# Autodesk Inventor assembly: roller
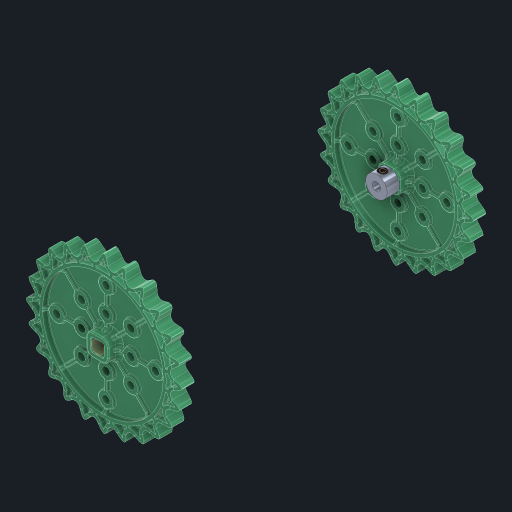
[picture p0: Inventor's stored thumbnail of the model, 512x512]
Saved by Autodesk Inventor 2024 (Build 280153000, 153)
## iProperties
Created: 2023-08-21
Part Number: roller
Document SubType Name: Assembly
Designer: Averey
Author: Averey
## Documents named in this file (4)
- C:\Users\Averey\Documents\vex\cad\scrap_v0.1\intake\roller.iam
- C:\Users\Averey\Documents\vex\cad\VEX-CAD-Inventor-1.41\Motion\Sprockets\9P Sprocket\9P 24T Sprocket, No Insert.iam
- C:\Users\Averey\Documents\vex\cad\VEX-CAD-Inventor-1.41\Motion\Sprockets\9P Sprocket.iam
- C:\Users\Averey\Documents\vex\cad\VEX-CAD-Inventor-1.41\Motion\Shaft LS\Shaft Collar ipts\Shaft Collar Set Screw.ipt
## Components (4 placed, 2 different names)
1. 9P 24T Sprocket, No Insert:1 [sub-assembly] — Insert:1, Insert:2
2. 9P 24T Sprocket, No Insert:2 [sub-assembly] — Insert:1, Insert:3
3. Shaft Collar Set Screw:1 — Insert:2
4. Shaft Collar Set Screw:2 — Insert:3
## Relationships (3: Insert 3)
- Insert:1 (136.525 mm): 9P 24T Sprocket, No Insert:1 ↔ 9P 24T Sprocket, No Insert:2
- Insert:2: 9P 24T Sprocket, No Insert:1 ↔ Shaft Collar Set Screw:1
- Insert:3: 9P 24T Sprocket, No Insert:2 ↔ Shaft Collar Set Screw:2
